# Autodesk Inventor assembly: Assembly1
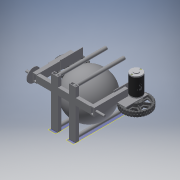
[picture p0: Inventor's stored thumbnail of the model, 180x180]
Saved by Autodesk Inventor 2016 SP1 (Build 200210100, 210)
## iProperties
Created: 2016-01-28
Part Number: Assembly1
Document SubType Name: Assembly
Designer: bbier
Author: bbier
## Documents named in this file (13)
- C:\snobotics\CAD-Development\robSteele\SnoBotics2016\Brian Bierman\2015-02-05\x\Assembly1.iam
- C:\snobotics\CAD-Development\robSteele\SnoBotics2016\Brian Bierman\2015-02-05\x\snoBackstop.ipt
- C:\snobotics\CAD-Development\robSteele\SnoBotics2016\Brian Bierman\2015-02-05\x\snoRail.ipt
- C:\snobotics\CAD-Development\robSteele\SnoBotics2016\Brian Bierman\2015-02-05\x\motorBracketLeft.ipt
- C:\snobotics\CAD-Development\robSteele\SnoBotics2016\Brian Bierman\2015-02-05\x\motorBracketRight.ipt
- C:\snobotics\CAD-Development\robSteele\SnoBotics2016\Brian Bierman\2015-02-05\x\6 wheel Rev 4.ipt
- C:\snobotics\CAD-Development\robSteele\SnoBotics2016\Brian Bierman\2015-02-05\x\boulder.ipt
- C:\snobotics\CAD-Development\robSteele\SnoBotics2016\Brian Bierman\2015-02-05\x\snoRiser.ipt
- C:\snobotics\CAD-Development\robSteele\SnoBotics2016\Brian Bierman\2015-02-05\x\snoRoundRail.ipt
- C:\snobotics\CAD-Development\robSteele\SnoBotics2016\Brian Bierman\2015-02-05\x\snoPivotChannel.ipt
- C:\snobotics\CAD-Development\robSteele\SnoBotics2016\Brian Bierman\2015-02-05\x\217-3371-STEP.ipt
- C:\snobotics\CAD-Development\robSteele\SnoBotics2016\Brian Bierman\2015-02-05\x\sprocket.ipt
- C:\snobotics\CAD-Development\robSteele\SnoBotics2016\AM Parts\MOT_CIM-Motor_217-2000_MIR7.iam
## Components (20 placed, 12 different names)
1. snoBackstop:1 — Flush:1, Flush:3, Mate:19, Mate:20, Mate:21, Flush:9, Flush:10, Flush:11, Flush:12, Flush:25
2. snoRail:1 — Flush:1, Mate:5, Mate:6, Flush:6, Angle:3, Angle:5, Mate:20, Flush:9, Flush:13, Mate:28, Mate:29, Flush:26
3. snoRail:2 — Flush:3, Mate:3, Mate:4, Flush:5, Mate:21, Flush:10, Flush:14, Mate:30, Mate:31, Flush:27
4. motorBracketLeft:1 — Mate:5, Mate:6, Flush:6, Mate:16, Mate:35, Mate:36, Insert:1
5. motorBracketRight:1 — Mate:3, Mate:4, Flush:5, Mate:14, Mate:32, Mate:33
6. 6 wheel Rev 4:1 — Mate:16, Mate:17, Angle:1, Mate:37
7. 6 wheel Rev 4:2 — Mate:14, Mate:18, Angle:2, Mate:34
8. boulder:1 — Tangent:1, Tangent:2, Tangent:3
9. snoRiser:1 — Flush:12, Flush:14, Flush:15, Mate:23, Angle:7, Mate:24, Angle:8, Angle:10, Angle:13, Mate:27, Angle:15, Angle:16, Flush:22, Angle:22, Flush:23, Flush:25
10. snoRiser:2 — Flush:11, Flush:13, Flush:15, Mate:25, Angle:9, Angle:11, Angle:12, Angle:14, Flush:18, Mate:26, Angle:19, Angle:20, Angle:21, Flush:21, Angle:23, Flush:24
11. snoRoundRail:1 — Mate:23, Tangent:4, Tangent:5, Tangent:7, Tangent:10
12. snoRoundRail:2 — Mate:25, Tangent:6, Tangent:8, Tangent:9, Tangent:11
13. snoRoundRail:3 — Mate:26, Tangent:16, Tangent:17, Tangent:18, Tangent:20
14. snoRoundRail:4 — Mate:27, Tangent:12, Tangent:13, Tangent:15, Tangent:19
15. snoPivotChannel:1 — Mate:30, Mate:31, Flush:27, Mate:38, Mate:39
16. snoPivotChannel:2 — Mate:28, Mate:29, Flush:26
17. 217-3371-STEP:1 — Mate:32, Mate:33, Mate:34
18. 217-3371-STEP:2 — Mate:35, Mate:36, Mate:37
19. sprocket:1 — Mate:38, Mate:39
20. MOT_CIM-Motor_217-2000_MIR7:2 [sub-assembly] — Insert:1
## Relationships (92: Mate 29, Angle 22, Flush 21, Tangent 19, Insert 1)
- Flush:1: snoBackstop:1 ↔ snoRail:1
- Flush:3: snoBackstop:1 ↔ snoRail:2
- Mate:3: snoRail:2 ↔ motorBracketRight:1
- Mate:4: snoRail:2 ↔ motorBracketRight:1
- Mate:5: snoRail:1 ↔ motorBracketLeft:1
- Mate:6: snoRail:1 ↔ motorBracketLeft:1
- Flush:5 (-64.008 mm): snoRail:2 ↔ motorBracketRight:1
- Flush:6 (-64.008 mm): snoRail:1 ↔ motorBracketLeft:1
- Mate:14 (3.175 mm): motorBracketRight:1 ↔ 6 wheel Rev 4:2
- Mate:16 (3.175 mm): motorBracketLeft:1 ↔ 6 wheel Rev 4:1
- Mate:17: 6 wheel Rev 4:1
- Angle:1 (0 deg): 6 wheel Rev 4:1
- Mate:18: 6 wheel Rev 4:2
- Angle:2 (0 deg): 6 wheel Rev 4:2
- Flush:7
- Mate:19: snoBackstop:1
- Angle:3 (0 deg): snoRail:1
- Angle:4 (0 deg)
- Tangent:1: boulder:1
- Angle:5 (0 deg): snoRail:1
- Tangent:2: boulder:1
- Angle:6 (0 deg)
- Tangent:3: boulder:1
- Flush:8 (123.825 mm)
- Mate:20: snoBackstop:1 ↔ snoRail:1
- Mate:21: snoBackstop:1 ↔ snoRail:2
- Mate:22 (-123.825 mm)
- Flush:9: snoBackstop:1 ↔ snoRail:1
- Flush:10: snoBackstop:1 ↔ snoRail:2
- Flush:11: snoBackstop:1 ↔ snoRiser:2
- Flush:12: snoBackstop:1 ↔ snoRiser:1
- Flush:13 (101.6 mm): snoRail:1 ↔ snoRiser:2
- Flush:14 (101.6 mm): snoRail:2 ↔ snoRiser:1
- Flush:15: snoRiser:1 ↔ snoRiser:2
- Mate:23: snoRiser:1 ↔ snoRoundRail:1
- Angle:7 (0 deg): snoRiser:1
- Tangent:4: snoRoundRail:1
- Mate:24 (-28.575 mm): snoRiser:1
- Mate:25: snoRiser:2 ↔ snoRoundRail:2
- Angle:8 (0 deg): snoRiser:1
- Tangent:5: snoRoundRail:1
- Angle:9 (0 deg): snoRiser:2
- Tangent:6: snoRoundRail:2
- Angle:10 (0 deg): snoRiser:1
- Tangent:7: snoRoundRail:1
- Angle:11 (0 deg): snoRiser:2
- Tangent:8: snoRoundRail:2
- Angle:12 (0 deg): snoRiser:2
- Tangent:9: snoRoundRail:2
- Angle:13 (0 deg): snoRiser:1
- Tangent:10: snoRoundRail:1
- Angle:14 (0 deg): snoRiser:2
- Tangent:11: snoRoundRail:2
- Flush:18 (9.525 mm): snoRiser:2
- Mate:26: snoRiser:2 ↔ snoRoundRail:3
- Mate:27: snoRiser:1 ↔ snoRoundRail:4
- Angle:15 (0 deg): snoRiser:1
- Tangent:12: snoRoundRail:4
- Angle:16 (0 deg): snoRiser:1
- Tangent:13: snoRoundRail:4
- Angle:18 (0 deg)
- Tangent:15: snoRoundRail:4
- Angle:19 (0 deg): snoRiser:2
- Tangent:16: snoRoundRail:3
- Angle:20 (0 deg): snoRiser:2
- Tangent:17: snoRoundRail:3
- Angle:21 (0 deg): snoRiser:2
- Tangent:18: snoRoundRail:3
- Flush:21 (9.525 mm): snoRiser:2
- Flush:22 (9.525 mm): snoRiser:1
- Angle:22 (0 deg): snoRiser:1
- Tangent:19: snoRoundRail:4
- Angle:23 (0 deg): snoRiser:2
- Tangent:20: snoRoundRail:3
- Flush:23 (3.175 mm): snoRiser:1
- Flush:24 (3.175 mm): snoRiser:2
- Flush:25 (-184.7342 mm): snoBackstop:1 ↔ snoRiser:1
- Mate:28: snoRail:1 ↔ snoPivotChannel:2
- Mate:29: snoRail:1 ↔ snoPivotChannel:2
- Flush:26: snoRail:1 ↔ snoPivotChannel:2
- Mate:30: snoRail:2 ↔ snoPivotChannel:1
- Mate:31: snoRail:2 ↔ snoPivotChannel:1
- Flush:27: snoRail:2 ↔ snoPivotChannel:1
- Mate:32: motorBracketRight:1 ↔ 217-3371-STEP:1
- Mate:33: motorBracketRight:1 ↔ 217-3371-STEP:1
- Mate:34: 6 wheel Rev 4:2 ↔ 217-3371-STEP:1
- Mate:35: motorBracketLeft:1 ↔ 217-3371-STEP:2
- Mate:36: motorBracketLeft:1 ↔ 217-3371-STEP:2
- Mate:37: 6 wheel Rev 4:1 ↔ 217-3371-STEP:2
- Mate:38: snoPivotChannel:1 ↔ sprocket:1
- Mate:39 (6.35 mm): snoPivotChannel:1 ↔ sprocket:1
- Insert:1: motorBracketLeft:1 ↔ MOT_CIM-Motor_217-2000_MIR7:2
